# Autodesk Inventor assembly: arm_gesamt
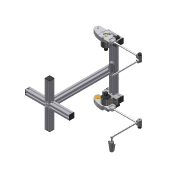
[picture p0: Inventor's stored thumbnail of the model, 180x180]
Saved by Autodesk Inventor 2021.4 (Build 254397000, 397)
## iProperties
Created: 2020-04-21
Part Number: arm_gesamt
Material: Generisch
Document SubType Name: Assembly
Designer: Alex
Mass: 5144.6 g
Surface Area: 14223.5 cm^2
Volume: 1845.1 cm^3
Density: 2.78825 g/cm^3
Author: Alex
## Documents named in this file (8)
- C:\Users\alexw\Documents\Inventor\Projects\03_CurrentProjects\MasterThesis\TrainingConsol_220422\Workgroups\Workgroup\arm_gesamt.iam
- C:\Users\alexw\Documents\Inventor\Projects\03_CurrentProjects\MasterThesis\TrainingConsol_220422\Workgroups\Workgroup\Gimbal_v2.iam
- C:\Users\alexw\Documents\Inventor\Projects\03_CurrentProjects\MasterThesis\TrainingConsol_220422\Workgroups\Workgroup\Arm_right_v3.iam
- C:\Users\alexw\Documents\Inventor\Projects\03_CurrentProjects\MasterThesis\TrainingConsol_220422\Workgroups\Workgroup\MTM_itemFrame.iam
- C:\Users\alexw\Documents\Inventor\Projects\03_CurrentProjects\MasterThesis\TrainingConsol_220422\Workgroups\Workgroup\Shoulder_Pitch_Assembly.iam
- C:\Users\alexw\Documents\Inventor\Projects\03_CurrentProjects\MasterThesis\TrainingConsol_220422\Workgroups\Workgroup\Arm_left_v3.iam
- C:\Users\alexw\Documents\Inventor\Projects\03_CurrentProjects\MasterThesis\TrainingConsol_220422\Workgroups\Workgroup\ContentCenter\en-US\ISO 10642(1)\ISO 10642 - M8x25.ipt
- C:\Users\alexw\Documents\Inventor\Projects\03_CurrentProjects\MasterThesis\TrainingConsol_220422\Workgroups\Workgroup\ContentCenter\en-US\ISO 4762(2)\ISO 4762 - M4 x 10ISO.ipt
## Components (10 placed, 7 different names)
1. Gimbal_v2:2 [sub-assembly] — Ball:2, Angle:7, Angle:8
2. Arm_right_v3:1 [sub-assembly] — Mate:676, Mate:677, Mate:681, Ball:2, q1_right, Angle:7, Angle:8
3. MTM_itemFrame:1 [sub-assembly] — Flush:91, Flush:92, Flush:93, Flush:94, Flush:95, Mate:672, Mate:673, Flush:96, Flush:97, Mate:674, Mate:675, q1_left, q1_right
4. Shoulder_Pitch_Assembly:1 [sub-assembly] — Flush:94, Flush:95, Mate:672, Mate:673, Mate:678, Mate:679
5. Shoulder_Pitch_Assembly:2 [sub-assembly] — Flush:96, Flush:97, Mate:674, Mate:675, Mate:676, Mate:677
6. Arm_left_v3:1 [sub-assembly] — Mate:678, Mate:679, Mate:680, Mate:682, Mate:683, Ball:1, q1_left, Angle:5, Angle:6
7. ISO 10642 M8x25:1 — Mate:680
8. ISO 10642 M8x25:2 — Mate:681
9. Gimbal_v2:3 [sub-assembly] — Ball:1, Angle:5, Angle:6
10. ISO 4762 M4 x 10:1 — Mate:682, Mate:683
## Relationships (28: Mate 13, Flush 7, Angle 6, BallJoint 2)
- Passend:305 [Mate]
- Flush:91: MTM_itemFrame:1
- Flush:92: MTM_itemFrame:1
- Flush:93: MTM_itemFrame:1
- Flush:94: MTM_itemFrame:1 ↔ Shoulder_Pitch_Assembly:1
- Flush:95: MTM_itemFrame:1 ↔ Shoulder_Pitch_Assembly:1
- Mate:672: MTM_itemFrame:1 ↔ Shoulder_Pitch_Assembly:1
- Mate:673: MTM_itemFrame:1 ↔ Shoulder_Pitch_Assembly:1
- Flush:96: MTM_itemFrame:1 ↔ Shoulder_Pitch_Assembly:2
- Flush:97: MTM_itemFrame:1 ↔ Shoulder_Pitch_Assembly:2
- Mate:674: MTM_itemFrame:1 ↔ Shoulder_Pitch_Assembly:2
- Mate:675: MTM_itemFrame:1 ↔ Shoulder_Pitch_Assembly:2
- Mate:676: Arm_right_v3:1 ↔ Shoulder_Pitch_Assembly:2
- Mate:677: Arm_right_v3:1 ↔ Shoulder_Pitch_Assembly:2
- Mate:678: Shoulder_Pitch_Assembly:1 ↔ Arm_left_v3:1
- Mate:679: Shoulder_Pitch_Assembly:1 ↔ Arm_left_v3:1
- Mate:680: Arm_left_v3:1 ↔ ISO 10642 M8x25:1
- Mate:681: Arm_right_v3:1 ↔ ISO 10642 M8x25:2
- Mate:682: Arm_left_v3:1 ↔ ISO 4762 M4 x 10:1
- Mate:683: Arm_left_v3:1 ↔ ISO 4762 M4 x 10:1
- Ball:1: Arm_left_v3:1 ↔ Gimbal_v2:3
- Ball:2: Gimbal_v2:2 ↔ Arm_right_v3:1
- q1_left [Angle] (0 deg): MTM_itemFrame:1 ↔ Arm_left_v3:1
- q1_right [Angle] (0 deg): Arm_right_v3:1 ↔ MTM_itemFrame:1
- Angle:5 (0 deg): Arm_left_v3:1 ↔ Gimbal_v2:3
- Angle:6 (0 deg): Arm_left_v3:1 ↔ Gimbal_v2:3
- Angle:7 (0 deg): Gimbal_v2:2 ↔ Arm_right_v3:1
- Angle:8 (0 deg): Gimbal_v2:2 ↔ Arm_right_v3:1
